# Autodesk Inventor assembly: lockingMechanismV01
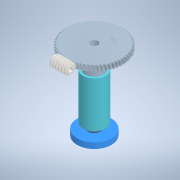
[picture p0: Inventor's stored thumbnail of the model, 180x180]
Saved by Autodesk Inventor 2021.1 (Build 251245000, 245)
## iProperties
Created: 2020-08-16
Part Number: lockingMechanismV01
Document SubType Name: Assembly
Designer: robst
Author: robst
## Documents named in this file (4)
- C:\git\CAD-Development\robSteele\ShapeWays\TelescopeProjects\TelescopeMount\BobSteeleLockingMechanism\lockingMechanismV01.iam
- C:\git\CAD-Development\robSteele\ShapeWays\TelescopeProjects\TelescopeMount\BobSteeleLockingMechanism\outerShell.ipt
- C:\git\CAD-Development\robSteele\ShapeWays\TelescopeProjects\TelescopeMount\BobSteeleLockingMechanism\handle.ipt
- C:\git\CAD-Development\robSteele\ShapeWays\TelescopeProjects\TelescopeMount\ForkMountWithCelestronTubeConnector\Design Accelerator\Worm Gears2.iam
## Components (3 placed, 3 different names)
1. outerShell:1 — Insert:1, Insert:2
2. handle:1 — Insert:1
3. Worm Gears:1 [sub-assembly] — Insert:2
## Relationships (2: Insert 2)
- Insert:1 (12.7 mm): outerShell:1 ↔ handle:1
- Insert:2: outerShell:1 ↔ Worm Gears:1
